# Autodesk Inventor assembly: Shoulder_support_assembly
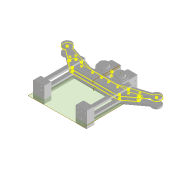
[picture p0: Inventor's stored thumbnail of the model, 180x180]
Saved by Autodesk Inventor 2022 (Build 260153000, 153)
## iProperties
Created: 2022-08-23
Part Number: Shoulder_support_assembly
Document SubType Name: Assembly
Designer: dell
Mass: 215.1 g
Surface Area: 1120.32 cm^2
Volume: 215.1 cm^3
Author: dell
## Documents named in this file (9)
- D:\xxxx\Uni\Part IV\MECHENG_700\Part_IV_project_CAD\Bird_skeleton_prototypes\Wing_drone_V1\Bird_wing_V2\Wing_shoulder\Shoulder_support_assembly.iam
- D:\xxxx\Uni\Part IV\MECHENG_700\Part_IV_project_CAD\Bird_skeleton_prototypes\Wing_drone_V1\Bird_wing_V2\Wing_shoulder\Vertical_bar.ipt
- D:\xxxx\Uni\Part IV\MECHENG_700\Part_IV_project_CAD\Bird_skeleton_prototypes\Wing_drone_V1\Bird_wing_V2\Wing_shoulder\Bar_connection_assembly.iam
- D:\xxxx\Uni\Part IV\MECHENG_700\Part_IV_project_CAD\Bird_skeleton_prototypes\Wing_drone_V1\Bird_wing_V2\Wing_shoulder\Horizontal_bar_V2.ipt
- D:\xxxx\Uni\Part IV\MECHENG_700\Part_IV_project_CAD\Bird_skeleton_prototypes\Wing_drone_V1\Bird_wing_V2\Motor_pulley_assembly.iam
- D:\xxxx\Uni\Part IV\MECHENG_700\Part_IV_project_CAD\Bird_skeleton_prototypes\Wing_drone_V1\Bird_wing_V2\Wing_shoulder\Horizontal_bar_support_V2.ipt
- D:\xxxx\Uni\Part IV\MECHENG_700\Part_IV_project_CAD\Bird_skeleton_prototypes\Wing_drone_V1\Bird_wing_V2\Wing_shoulder\Horizontal_bar_spacer.ipt
- D:\xxxx\Uni\Part IV\MECHENG_700\Part_IV_project_CAD\Bird_skeleton_prototypes\Wing_drone_V1\Bird_wing_V2\Wing_shoulder\Horizontal_bar_p2_V2.ipt
- D:\xxxx\Uni\Part IV\MECHENG_700\Part_IV_project_CAD\Bird_skeleton_prototypes\Wing_drone_V1\Bird_wing_V2\Wing_shoulder\Horizontal_bar_spacer_small.ipt
## Components (25 placed, 8 different names)
1. Vertical_bar:1 — Flush:1, Flush:4, Mate:5, Symmetry:1, Mate:12
2. Vertical_bar:2 — Flush:1, Flush:4, Mate:9, Mate:10, Flush:8, Mate:12, Mate:13, Mate:17
3. Vertical_bar:3 — Flush:2, Flush:3, Symmetry:1, Mate:7, Mate:8, Flush:7, Mate:15, Mate:18
4. Vertical_bar:4 — Flush:2, Flush:3, Mate:5, Mate:16, Mate:26, Mate:27
5. Bar_connection_assembly:1 [sub-assembly] — Mate:9, Mate:10, Flush:8, Mate:48, Mate:49
6. Bar_connection_assembly:2 [sub-assembly] — Mate:7, Mate:8, Flush:7, Mate:50, Mate:51
7. Horizontal_bar_V2:1 — Mate:13, Mate:15, Mate:16, Mate:17, Mate:18, Mate:19, Mate:20, Mate:21, Mate:23, Mate:24, Mate:25, Mate:28, Mate:30, Mate:52, Mate:53, Mate:54, Mate:55
8. Motor_pulley_assembly:3 [sub-assembly] — Mate:19, Mate:20, Mate:21, Mate:22
9. Motor_pulley_assembly:4 [sub-assembly] — Mate:23, Mate:24, Mate:25
10. Horizontal_bar_support_V2:2 — Mate:26, Mate:27, Mate:29, Mate:31, Mate:41, Mate:42, Mate:43, Mate:56, Mate:57, Mate:58, Mate:59, Mate:60, Mate:61, Mate:62, Mate:63, Mate:64, Mate:65, Mate:66, Mate:67
11. Horizontal_bar_spacer:4 — Mate:30, Mate:31
12. Horizontal_bar_spacer:5 — Mate:28, Mate:29
13. Horizontal_bar_p2_V2:1 — Mate:41, Mate:42, Mate:43, Mate:44, Mate:45, Mate:46, Mate:47
14. Horizontal_bar_spacer_small:1 — Mate:44, Mate:45
15. Horizontal_bar_spacer_small:2 — Mate:46, Mate:47
16. Vertical_bar:5 — Mate:48, Mate:49
17. Vertical_bar:6 — Mate:50, Mate:51
18. Horizontal_bar_spacer:6 — Mate:54, Mate:55
19. Horizontal_bar_spacer:7 — Mate:52, Mate:53
20. Horizontal_bar_spacer_small:3 — Mate:56, Mate:57
21. Horizontal_bar_spacer_small:4 — Mate:58, Mate:59
22. Horizontal_bar_spacer_small:5 — Mate:60, Mate:61
23. Horizontal_bar_spacer_small:6 — Mate:62, Mate:63
24. Horizontal_bar_spacer_small:7 — Mate:64, Mate:65
25. Horizontal_bar_spacer_small:8 — Mate:66, Mate:67
## Relationships (58: Mate 51, Flush 6, Symmetry 1)
- Flush:1: Vertical_bar:1 ↔ Vertical_bar:2
- Flush:2: Vertical_bar:3 ↔ Vertical_bar:4
- Flush:3: Vertical_bar:3 ↔ Vertical_bar:4
- Flush:4: Vertical_bar:1 ↔ Vertical_bar:2
- Mate:5 (120 mm): Vertical_bar:1 ↔ Vertical_bar:4
- Symmetry:1: Vertical_bar:1 ↔ Vertical_bar:3
- Mate:7: Vertical_bar:3 ↔ Bar_connection_assembly:2
- Mate:8: Vertical_bar:3 ↔ Bar_connection_assembly:2
- Flush:7: Vertical_bar:3 ↔ Bar_connection_assembly:2
- Mate:9: Vertical_bar:2 ↔ Bar_connection_assembly:1
- Mate:10: Vertical_bar:2 ↔ Bar_connection_assembly:1
- Flush:8: Vertical_bar:2 ↔ Bar_connection_assembly:1
- Mate:12 (5 mm): Vertical_bar:1 ↔ Vertical_bar:2
- Mate:13: Vertical_bar:2 ↔ Horizontal_bar_V2:1
- Mate:15: Vertical_bar:3 ↔ Horizontal_bar_V2:1
- Mate:16: Vertical_bar:4 ↔ Horizontal_bar_V2:1
- Mate:17: Vertical_bar:2 ↔ Horizontal_bar_V2:1
- Mate:18: Vertical_bar:3 ↔ Horizontal_bar_V2:1
- Mate:19: Horizontal_bar_V2:1 ↔ Motor_pulley_assembly:3
- Mate:20: Horizontal_bar_V2:1 ↔ Motor_pulley_assembly:3
- Mate:21: Horizontal_bar_V2:1 ↔ Motor_pulley_assembly:3
- Mate:22: Motor_pulley_assembly:3
- Mate:23: Horizontal_bar_V2:1 ↔ Motor_pulley_assembly:4
- Mate:24: Horizontal_bar_V2:1 ↔ Motor_pulley_assembly:4
- Mate:25: Horizontal_bar_V2:1 ↔ Motor_pulley_assembly:4
- Mate:26: Vertical_bar:4 ↔ Horizontal_bar_support_V2:2
- Mate:27: Vertical_bar:4 ↔ Horizontal_bar_support_V2:2
- Mate:28: Horizontal_bar_V2:1 ↔ Horizontal_bar_spacer:5
- Mate:29: Horizontal_bar_support_V2:2 ↔ Horizontal_bar_spacer:5
- Mate:30: Horizontal_bar_V2:1 ↔ Horizontal_bar_spacer:4
- Mate:31: Horizontal_bar_support_V2:2 ↔ Horizontal_bar_spacer:4
- Mate:41 (4.2 mm): Horizontal_bar_support_V2:2 ↔ Horizontal_bar_p2_V2:1
- Mate:42: Horizontal_bar_support_V2:2 ↔ Horizontal_bar_p2_V2:1
- Mate:43: Horizontal_bar_support_V2:2 ↔ Horizontal_bar_p2_V2:1
- Mate:44: Horizontal_bar_p2_V2:1 ↔ Horizontal_bar_spacer_small:1
- Mate:45: Horizontal_bar_p2_V2:1 ↔ Horizontal_bar_spacer_small:1
- Mate:46: Horizontal_bar_p2_V2:1 ↔ Horizontal_bar_spacer_small:2
- Mate:47: Horizontal_bar_p2_V2:1 ↔ Horizontal_bar_spacer_small:2
- Mate:48: Bar_connection_assembly:1 ↔ Vertical_bar:5
- Mate:49 (0.1 mm): Bar_connection_assembly:1 ↔ Vertical_bar:5
- Mate:50: Bar_connection_assembly:2 ↔ Vertical_bar:6
- Mate:51 (0.1 mm): Bar_connection_assembly:2 ↔ Vertical_bar:6
- Mate:52: Horizontal_bar_V2:1 ↔ Horizontal_bar_spacer:7
- Mate:53: Horizontal_bar_V2:1 ↔ Horizontal_bar_spacer:7
- Mate:54: Horizontal_bar_V2:1 ↔ Horizontal_bar_spacer:6
- Mate:55: Horizontal_bar_V2:1 ↔ Horizontal_bar_spacer:6
- Mate:56: Horizontal_bar_support_V2:2 ↔ Horizontal_bar_spacer_small:3
- Mate:57: Horizontal_bar_support_V2:2 ↔ Horizontal_bar_spacer_small:3
- Mate:58: Horizontal_bar_support_V2:2 ↔ Horizontal_bar_spacer_small:4
- Mate:59: Horizontal_bar_support_V2:2 ↔ Horizontal_bar_spacer_small:4
- Mate:60: Horizontal_bar_support_V2:2 ↔ Horizontal_bar_spacer_small:5
- Mate:61: Horizontal_bar_support_V2:2 ↔ Horizontal_bar_spacer_small:5
- Mate:62: Horizontal_bar_support_V2:2 ↔ Horizontal_bar_spacer_small:6
- Mate:63: Horizontal_bar_support_V2:2 ↔ Horizontal_bar_spacer_small:6
- Mate:64: Horizontal_bar_support_V2:2 ↔ Horizontal_bar_spacer_small:7
- Mate:65: Horizontal_bar_support_V2:2 ↔ Horizontal_bar_spacer_small:7
- Mate:66: Horizontal_bar_support_V2:2 ↔ Horizontal_bar_spacer_small:8
- Mate:67: Horizontal_bar_support_V2:2 ↔ Horizontal_bar_spacer_small:8
